# Autodesk Inventor assembly: Mechanical Pencil
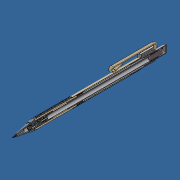
[picture p0: Inventor's stored thumbnail of the model, 180x180]
Saved by Autodesk Inventor 2022.4 (Build 264492010, 492A)
## iProperties
Created: 2008-09-23
Part Number: Mechanical Pencil
Document SubType Name: Assembly
Designer: Mark Flayler
Mass: 17.6894 g
Surface Area: 137.126 cm^2
Volume: 3.92401 cm^3
Density: 4.50798 g/cm^3
CN_MASS: 0.02
Author: Mark Flayler
## Documents named in this file (14)
- U:\Inventor 2022 Training\_Designer Training\Inventor 2022 - Advanced Assembly\Practice Files\Mechanical_Pencil_Simplify\Mechanical Pencil.iam
- U:\Inventor 2022 Training\_Designer Training\Inventor 2022 - Advanced Assembly\Practice Files\Mechanical_Pencil_Simplify\Clip.ipt
- U:\Inventor 2022 Training\_Designer Training\Inventor 2022 - Advanced Assembly\Practice Files\Mechanical_Pencil_Simplify\Cone.ipt
- U:\Inventor 2022 Training\_Designer Training\Inventor 2022 - Advanced Assembly\Practice Files\Mechanical_Pencil_Simplify\Coupling.ipt
- U:\Inventor 2022 Training\_Designer Training\Inventor 2022 - Advanced Assembly\Practice Files\Mechanical_Pencil_Simplify\Dispenser Ring.ipt
- U:\Inventor 2022 Training\_Designer Training\Inventor 2022 - Advanced Assembly\Practice Files\Mechanical_Pencil_Simplify\Dispenser.ipt
- U:\Inventor 2022 Training\_Designer Training\Inventor 2022 - Advanced Assembly\Practice Files\Mechanical_Pencil_Simplify\Eraser Cap.ipt
- U:\Inventor 2022 Training\_Designer Training\Inventor 2022 - Advanced Assembly\Practice Files\Mechanical_Pencil_Simplify\Eraser.ipt
- U:\Inventor 2022 Training\_Designer Training\Inventor 2022 - Advanced Assembly\Practice Files\Mechanical_Pencil_Simplify\Lead Guide.ipt
- U:\Inventor 2022 Training\_Designer Training\Inventor 2022 - Advanced Assembly\Practice Files\Mechanical_Pencil_Simplify\Shaft Dispenser.ipt
- U:\Inventor 2022 Training\_Designer Training\Inventor 2022 - Advanced Assembly\Practice Files\Mechanical_Pencil_Simplify\Spring.ipt
- U:\Inventor 2022 Training\_Designer Training\Inventor 2022 - Advanced Assembly\Practice Files\Mechanical_Pencil_Simplify\Upper Shaft.ipt
- U:\Inventor 2022 Training\_Designer Training\Inventor 2022 - Advanced Assembly\Practice Files\Mechanical_Pencil_Simplify\Pencil Shaft.ipt
- U:\Inventor 2022 Training\_Designer Training\Inventor 2022 - Advanced Assembly\Practice Files\Mechanical_Pencil_Simplify\Housing.iam
## Components (13 placed, 13 different names)
1. Pencil Shaft:1 — Insert:2, Insert:3, Insert:4
2. Clip:1 — Mate:1, Mate:2, Mate:3
3. Cone:1 — Insert:1, Insert:5, Insert:6, Insert:9
4. Coupling:1 — Insert:7
5. Dispenser Ring:1 — Insert:5
6. Dispenser:1 — Insert:6, Insert:7, Mate:4
7. Eraser Cap:1 — Insert:3
8. Eraser:1 — Insert:2
9. Lead Guide:1 — Insert:1
10. Shaft Dispenser:1 — Insert:9, Mate:5
11. Spring:1 — Mate:4, Mate:5
12. Upper Shaft:1 — Mate:1, Mate:2, Mate:3, Insert:4, Flush:1
13. Housing:1 [sub-assembly]
## Relationships (17: Insert 9, Mate 7, Flush 1)
- Mate:1: Clip:1 ↔ Upper Shaft:1
- Mate:2: Clip:1 ↔ Upper Shaft:1
- Insert:1 (-1 mm): Cone:1 ↔ Lead Guide:1
- Insert:2: Pencil Shaft:1 ↔ Eraser:1
- Insert:3: Pencil Shaft:1 ↔ Eraser Cap:1
- Mate:3: Clip:1 ↔ Upper Shaft:1
- Insert:4 (4 mm): Pencil Shaft:1 ↔ Upper Shaft:1
- Insert:5: Cone:1 ↔ Dispenser Ring:1
- Insert:6: Cone:1 ↔ Dispenser:1
- Insert:7: Coupling:1 ↔ Dispenser:1
- [Insert]: Cone:1 ↔ Housing:1
- Mate:4: Dispenser:1 ↔ Spring:1
- Insert:9: Cone:1 ↔ Shaft Dispenser:1
- Mate:5: Shaft Dispenser:1 ↔ Spring:1
- [Mate]: Upper Shaft:1 ↔ Housing:1
- [Mate]: Upper Shaft:1 ↔ Housing:1
- Flush:1: Upper Shaft:1
